# Autodesk Inventor assembly: AM14U2 Half Long
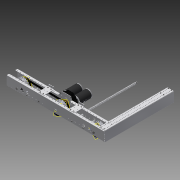
[picture p0: Inventor's stored thumbnail of the model, 180x180]
Saved by Autodesk Inventor 2015 SP1 (Build 190203100, 203)
## iProperties
Created: 2014-12-16
Part Number: AM14U2 Half Long
Document SubType Name: Assembly
Designer: Philip
Author: Philip
## Documents named in this file (18)
- C:\FRC_KOP_2015_Test\Drive Base\Parts\AM14U2 Half Long.iam
- C:\FRC_KOP_2015_Test\Drive Base\Parts\2014 KoP - 4 HiGrip and Double 42 HTD Pulley.iam
- C:\FRC_KOP_2015_Test\Drive Base\Parts\2014 KoP - 4 HiGrip and Single 42 HTD Pulley.iam
- C:\FRC_KOP_2015_Test\Drive Base\Parts\am-1305 500 Hex Spacer.ipt
- C:\FRC_KOP_2015_Test\Drive Base\Parts\Toughbox Mini L-Base.iam
- C:\FRC_KOP_2015_Test\Drive Base\Parts\FR8ZZ Hex Bearing.ipt
- C:\FRC_KOP_2015_Test\Drive Base\Parts\am-2951 AM14U2 Outside Sheet.ipt
- C:\FRC_KOP_2015_Test\Drive Base\Parts\am-2952 AM14U2 Inside Sheet.ipt
- C:\FRC_KOP_2015_Test\Drive Base\Parts\Churro 3375 and Screws.iam
- C:\FRC_KOP_2015_Test\Drive Base\Parts\spacer 0850 WashersUSA 13RS075054.ipt
- C:\FRC_KOP_2015_Test\Drive Base\Parts\spacer 0280 WashersUSA 13RS052001.ipt
- C:\FRC_KOP_2015_Test\Drive Base\Parts\Sheet Metal Front-Back.ipt
- C:\FRC_KOP_2015_Test\Drive Base\Parts\Churro cross link and Screws.iam
- C:\FRC_KOP_2015_Test\Drive Base\Parts\3-8-16 NyLock Nut - Mcm 95615A140_95615A140.ipt
- C:\FRC_KOP_2015_Test\Drive Base\Parts\10-32x0625 with nut.iam
- C:\FRC_KOP_2015_Test\Drive Base\Parts\am-2954 AM14U2 2x3 Hole Bracket.ipt
- C:\FRC_KOP_2015_Test\Drive Base\Parts\375-16 x 4.25 Hex Bolt_HFBOLT 0.375-16x2.5x1-C.ipt
- C:\FRC_KOP_2015_Test\Drive Base\Parts\5mm-15mm-170T Belt.ipt
## Components (46 placed, 46 different names)
1. 2014 KoP - 4 HiGrip and Double 42 HTD Pulley_3 [sub-assembly] — Mate:6, Flush:1, Angle:3, Mate:7, Mate:8, Mate:9
2. 2014 KoP - 4 HiGrip and Single 42 HTD Pulley_4 [sub-assembly] — Flush:1
3. 2014 KoP - 4 HiGrip and Single 42 HTD Pulley_5 [sub-assembly]
4. am-1305 500 Hex Spacer_6 — Mate:7, Mate:8, Angle:4, Mate:9
5. Toughbox Mini L-Base_7 [sub-assembly] — Insert:1, Insert:2, Mate:1, Mate:2, Mate:3, Angle:2, Angle:3
6. FR8ZZ Hex Bearing_8 — Mate:4, Mate:5, Angle:2, Angle:4
7. am-2951 AM14U2 Outside Sheet_9 — Mate:4, Mate:5, Insert:3, Insert:4, Insert:5, Insert:6, Insert:9, Angle:1
8. am-2952 AM14U2 Inside Sheet_10 — Insert:1, Insert:2, Mate:1, Mate:2, Mate:3, Insert:7, Insert:8, Mate:6
9. Churro 3375 and Screws_11 [sub-assembly]
10. Churro 3375 and Screws_12 [sub-assembly]
11. Churro 3375 and Screws_13 [sub-assembly]
12. Churro 3375 and Screws_14 [sub-assembly] — Insert:9, Angle:1
13. spacer 0850 WashersUSA 13RS075054_15
14. spacer 0280 WashersUSA 13RS052001_16
15. spacer 0850 WashersUSA 13RS075054_17
16. spacer 0280 WashersUSA 13RS052001_18
17. Sheet Metal Front-Back_19 — Insert:3, Insert:4
18. Churro cross link and Screws_20 [sub-assembly]
19. 3-8-16 NyLock Nut - Mcm 95615A140_95615A140_21
20. 10-32x0625 with nut_22 [sub-assembly]
21. 10-32x0625 with nut_23 [sub-assembly]
22. 10-32x0625 with nut_24 [sub-assembly]
23. 10-32x0625 with nut_25 [sub-assembly]
24. 10-32x0625 with nut_26 [sub-assembly]
25. 10-32x0625 with nut_27 [sub-assembly]
26. 10-32x0625 with nut_28 [sub-assembly]
27. 10-32x0625 with nut_29 [sub-assembly]
28. 10-32x0625 with nut_30 [sub-assembly]
29. 10-32x0625 with nut_31 [sub-assembly]
30. 10-32x0625 with nut_32 [sub-assembly]
31. 10-32x0625 with nut_33 [sub-assembly]
32. am-2954 AM14U2 2x3 Hole Bracket_34 — Insert:5, Insert:6, Insert:7, Insert:8
33. am-2954 AM14U2 2x3 Hole Bracket_35
34. 10-32x0625 with nut_36 [sub-assembly]
35. 10-32x0625 with nut_37 [sub-assembly]
36. 10-32x0625 with nut_38 [sub-assembly]
37. 10-32x0625 with nut_39 [sub-assembly]
38. 10-32x0625 with nut_40 [sub-assembly]
39. 10-32x0625 with nut_41 [sub-assembly]
40. 10-32x0625 with nut_42 [sub-assembly]
41. 10-32x0625 with nut_43 [sub-assembly]
42. 375-16 x 4.25 Hex Bolt_HFBOLT 0.375-16x2.5x1-C_44
43. 375-16 x 4.25 Hex Bolt_HFBOLT 0.375-16x2.5x1-C_45
44. 3-8-16 NyLock Nut - Mcm 95615A140_95615A140_46
45. 5mm-15mm-170T Belt_47
46. 5mm-15mm-170T Belt_48
## Relationships (23: Insert 9, Mate 9, Angle 4, Flush 1)
- Insert:1: Toughbox Mini L-Base_7 ↔ am-2952 AM14U2 Inside Sheet_10
- Insert:2: Toughbox Mini L-Base_7 ↔ am-2952 AM14U2 Inside Sheet_10
- Mate:1: Toughbox Mini L-Base_7 ↔ am-2952 AM14U2 Inside Sheet_10
- Mate:2: Toughbox Mini L-Base_7 ↔ am-2952 AM14U2 Inside Sheet_10
- Mate:3: Toughbox Mini L-Base_7 ↔ am-2952 AM14U2 Inside Sheet_10
- Mate:4: FR8ZZ Hex Bearing_8 ↔ am-2951 AM14U2 Outside Sheet_9
- Mate:5: FR8ZZ Hex Bearing_8 ↔ am-2951 AM14U2 Outside Sheet_9
- Insert:3: am-2951 AM14U2 Outside Sheet_9 ↔ Sheet Metal Front-Back_19
- Insert:4: am-2951 AM14U2 Outside Sheet_9 ↔ Sheet Metal Front-Back_19
- Insert:5: am-2951 AM14U2 Outside Sheet_9 ↔ am-2954 AM14U2 2x3 Hole Bracket_34
- Insert:6: am-2951 AM14U2 Outside Sheet_9 ↔ am-2954 AM14U2 2x3 Hole Bracket_34
- Insert:7: am-2952 AM14U2 Inside Sheet_10 ↔ am-2954 AM14U2 2x3 Hole Bracket_34
- Insert:8: am-2952 AM14U2 Inside Sheet_10 ↔ am-2954 AM14U2 2x3 Hole Bracket_34
- Insert:9: am-2951 AM14U2 Outside Sheet_9 ↔ Churro 3375 and Screws_14
- Angle:1 (0 deg): am-2951 AM14U2 Outside Sheet_9 ↔ Churro 3375 and Screws_14
- Angle:2 (0 deg): Toughbox Mini L-Base_7 ↔ FR8ZZ Hex Bearing_8
- Mate:6: 2014 KoP - 4 HiGrip and Double 42 HTD Pulley_3 ↔ am-2952 AM14U2 Inside Sheet_10
- Flush:1: 2014 KoP - 4 HiGrip and Double 42 HTD Pulley_3 ↔ 2014 KoP - 4 HiGrip and Single 42 HTD Pulley_4
- Angle:3 (0 deg): 2014 KoP - 4 HiGrip and Double 42 HTD Pulley_3 ↔ Toughbox Mini L-Base_7
- Mate:7: 2014 KoP - 4 HiGrip and Double 42 HTD Pulley_3 ↔ am-1305 500 Hex Spacer_6
- Mate:8: 2014 KoP - 4 HiGrip and Double 42 HTD Pulley_3 ↔ am-1305 500 Hex Spacer_6
- Angle:4 (0 deg): am-1305 500 Hex Spacer_6 ↔ FR8ZZ Hex Bearing_8
- Mate:9: 2014 KoP - 4 HiGrip and Double 42 HTD Pulley_3 ↔ am-1305 500 Hex Spacer_6
